# Autodesk Inventor assembly: Chain Z-Mount Unit
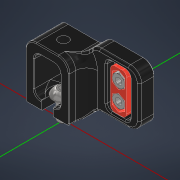
[picture p0: Inventor's stored thumbnail of the model, 180x180]
Saved by Autodesk Inventor 2022.2 (Build 262287010, 287A)
## iProperties
Created: 2022-03-23
Part Number: Chain Z-Mount Unit
Document SubType Name: Assembly
Designer: sleib
Author: sleib
## Documents named in this file (5)
- C:\Users\sleib\Projekte\Voron-2\CAD\Inventor\Chain Z-Mount Unit.iam
- C:\Users\sleib\Projekte\Voron-2\CAD\Inventor\Chain Z-Mount.ipt
- C:\Users\sleib\Projekte\Voron-2\CAD\Inventor\Chain Retainer-Bracket.ipt
- C:\Users\sleib\Projekte\Voron-2\CAD\Inventor\M3 Hexnut.ipt
- C:\Users\sleib\Projekte\Voron-2\CAD\Inventor\M5x10 BHCS.ipt
## Components (5 placed, 4 different names)
1. Chain Z-Mount:1 — Passend:1, Passend:2, Fluchtend:1, Passend:9, Passend:10, Tangential:1, Passend:11, Passend:12
2. Chain Retainer-Bracket:1 — Passend:3, Passend:4, Passend:7, Passend:8, Passend:9, Passend:10, Tangential:1
3. M3 Hexnut:1 — Passend:3, Fluchtend:2, Passend:6, Passend:7
4. M3 Hexnut:2 — Passend:4, Fluchtend:2, Passend:6, Passend:8
5. M5x10 BHCS:1 — Passend:11, Passend:12
## Relationships (14: Mate 11, Flush 2, Tangent 1)
- Passend:1 [Mate]: Chain Z-Mount:1
- Passend:2 [Mate]: Chain Z-Mount:1
- Fluchtend:1 [Flush] (-7.5 mm): Chain Z-Mount:1
- Passend:3 [Mate]: Chain Retainer-Bracket:1 ↔ M3 Hexnut:1
- Passend:4 [Mate]: Chain Retainer-Bracket:1 ↔ M3 Hexnut:2
- Fluchtend:2 [Flush]: M3 Hexnut:1 ↔ M3 Hexnut:2
- Passend:6 [Mate] (8 mm): M3 Hexnut:1 ↔ M3 Hexnut:2
- Passend:7 [Mate]: Chain Retainer-Bracket:1 ↔ M3 Hexnut:1
- Passend:8 [Mate]: Chain Retainer-Bracket:1 ↔ M3 Hexnut:2
- Passend:9 [Mate]: Chain Z-Mount:1 ↔ Chain Retainer-Bracket:1
- Passend:10 [Mate] (2 mm): Chain Z-Mount:1 ↔ Chain Retainer-Bracket:1
- Tangential:1: Chain Z-Mount:1 ↔ Chain Retainer-Bracket:1
- Passend:11 [Mate]: Chain Z-Mount:1 ↔ M5x10 BHCS:1
- Passend:12 [Mate]: Chain Z-Mount:1 ↔ M5x10 BHCS:1
